# Autodesk Inventor assembly: Intake Full Assembly
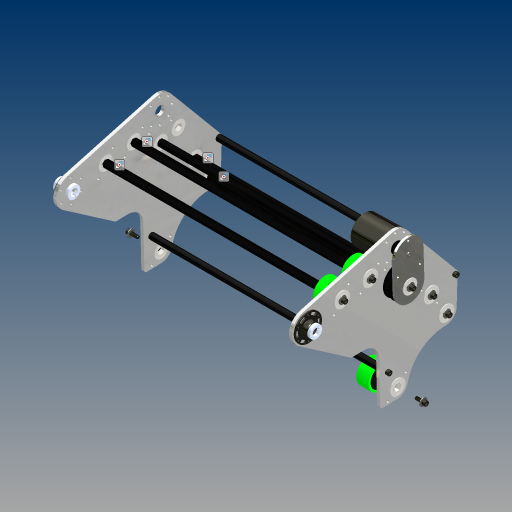
[picture p0: Inventor's stored thumbnail of the model, 512x512]
Saved by Autodesk Inventor 2024.3 (Build 283343000, 343)
## iProperties
Created: 2024-07-29
Part Number: Intake Full Assembly
Document SubType Name: Assembly
Designer: Kenji
Author: Kenji
## Documents named in this file (18)
- C:\Users\Kenji\Documents\GitHub\1622-2024-Summer-CAD-A-Thon\Intake\Intake Full Assembly.iam
- C:\Users\Kenji\Documents\GitHub\1622-2024-Summer-CAD-A-Thon\Intake\Intake Roller Plate.ipt
- C:\Users\Kenji\Documents\GitHub\1622-2024-Summer-CAD-A-Thon\COTS Library\Motion\Bearings\COTS_WCP-0783_1.125ODHexBearing.ipt
- C:\Users\Kenji\Documents\GitHub\1622-2024-Summer-CAD-A-Thon\Intake\Intake HexShaft 1.ipt
- C:\Users\Kenji\Documents\GitHub\1622-2024-Summer-CAD-A-Thon\COTS Library\Motion\Wheels\Compliant Wheels\2in compliant wheels\0.500in hex bore\COTS_am-3462_2indiameter_0.500inhexbore_durometer35A_CompliantWheel.ipt
- C:\Users\Kenji\Documents\GitHub\1622-2024-Summer-CAD-A-Thon\COTS Library\Motion\Wheels\Stealth Wheels\COTS_am-3155 2IN 500Hex Stealth Wheel.iam
- C:\Users\Kenji\Documents\GitHub\1622-2024-Summer-CAD-A-Thon\COTS Library\Structural Adapter\VersaHubs\COTS_217-2592_VersaHub.ipt
- C:\Users\Kenji\Documents\GitHub\1622-2024-Summer-CAD-A-Thon\Intake\Intake BeaterBar.ipt
- C:\Users\Kenji\Documents\GitHub\1622-2024-Summer-CAD-A-Thon\COTS Library\Fasteners\Bolts\Socket-Head\0.25-20\COTS_91251A539_Black-Oxide Alloy Steel Socket Head Screw (1).ipt
- C:\Users\Kenji\Documents\GitHub\1622-2024-Summer-CAD-A-Thon\COTS Library\Fasteners\Washers\COTS_90107A029_316 Stainless Steel Washer.ipt
- C:\Users\Kenji\Documents\GitHub\1622-2024-Summer-CAD-A-Thon\COTS Library\Fasteners\Shaft Collars\COTS_WCP-0799_0.5inchHexShaftCollar.ipt
- C:\Users\Kenji\Documents\GitHub\1622-2024-Summer-CAD-A-Thon\COTS Library\Motors\COTS_REV-21-1650-V1.1.ipt
- C:\Users\Kenji\Documents\GitHub\1622-2024-Summer-CAD-A-Thon\Intake\WCP-0076.ipt
- C:\Users\Kenji\Documents\GitHub\1622-2024-Summer-CAD-A-Thon\Intake\WCP-0990 (1).ipt
- C:\Users\Kenji\Documents\GitHub\1622-2024-Summer-CAD-A-Thon\Intake\WCP-0706.ipt
- C:\Users\Kenji\Documents\GitHub\1622-2024-Summer-CAD-A-Thon\Intake\WCP-0563.ipt
- C:\Users\Kenji\Documents\GitHub\1622-2024-Summer-CAD-A-Thon\Intake\Intake Hex Shaft 3.ipt
- C:\Users\Kenji\Documents\GitHub\1622-2024-Summer-CAD-A-Thon\Intake\Intake Pulley Cover 1.ipt
## Components (71 placed, 17 different names)
1. Intake Roller Plate:1 — Mate:293, Mate:294, Mate:295, Mate:296, Mate:297, Mate:298, Mate:299, Mate:302, Mate:303, Mate:304, Mate:306, Mate:307, Mate:308, Mate:310, Mate:311, Mate:312, Mate:313, Mate:314, Mate:315, Mate:316, Mate:317, Mate:318, Mate:319, Mate:320, Mate:321, Mate:364
2. Intake Roller Plate:2 — Mate:270, Mate:272, Mate:273, Mate:275, Mate:276, Mate:277, Mate:278, Mate:279, Mate:280, Mate:281, Mate:282, Mate:283, Mate:284, Mate:285, Mate:286, Mate:287, Mate:290, Mate:291, Mate:292, Mate:300, Mate:301, Mate:346, Mate:347, Mate:348
3. COTS_WCP-0783_1.125ODHexBearing:1 — Mate:25, Mate:276, Mate:283, Mate:329, Mate:340, Flush:10, Mate:355
4. COTS_WCP-0783_1.125ODHexBearing:2 — Mate:26, Mate:277, Mate:278, Mate:334, Mate:352, Mate:353
5. COTS_WCP-0783_1.125ODHexBearing:3 — Mate:272, Mate:280, Mate:332, Mate:337, Flush:11, Mate:358
6. COTS_WCP-0783_1.125ODHexBearing:4 — Mate:233, Mate:275, Mate:282, Mate:330, Mate:339, Flush:9, Mate:356
7. COTS_WCP-0783_1.125ODHexBearing:5 — Mate:270, Mate:271, Mate:279, Mate:333, Mate:336, Flush:12, Mate:357
8. COTS_WCP-0783_1.125ODHexBearing:6 — Mate:273, Mate:274, Mate:281, Mate:331, Mate:344, Mate:345
9. COTS_WCP-0783_1.125ODHexBearing:7 — Mate:135, Mate:319, Mate:320, Mate:326, Mate:360
10. COTS_WCP-0783_1.125ODHexBearing:8 — Mate:130, Mate:315, Mate:316, Mate:324, Mate:342, Mate:361
11. COTS_WCP-0783_1.125ODHexBearing:9 — Mate:134, Mate:317, Mate:318, Mate:325
12. COTS_WCP-0783_1.125ODHexBearing:10 — Mate:25, Mate:136, Mate:294, Mate:295, Mate:323, Mate:362
13. COTS_WCP-0783_1.125ODHexBearing:11 — Mate:26, Mate:132, Mate:144, Mate:293, Mate:321, Mate:328
14. COTS_WCP-0783_1.125ODHexBearing:12 — Mate:33, Mate:133, Mate:313, Mate:314, Mate:327, Mate:359
15. COTS_217-2592_VersaHub:2 — Mate:262, Mate:263, Mate:302, Mate:303, Mate:304, Mate:305
16. COTS_217-2592_VersaHub:3 — Mate:266, Mate:267, Mate:284, Mate:285, Mate:286
17. COTS_am-3462_2indiameter_0.500inhexbore_durometer35A_CompliantWheel:66 — Mate:136
18. COTS_am-3462_2indiameter_0.500inhexbore_durometer35A_CompliantWheel:24 — Mate:33, Mate:133
19. COTS_am-3462_2indiameter_0.500inhexbore_durometer35A_CompliantWheel:25 — Mate:134
20. COTS_am-3462_2indiameter_0.500inhexbore_durometer35A_CompliantWheel:53 — Mate:135
21. COTS_am-3462_2indiameter_0.500inhexbore_durometer35A_CompliantWheel:40 — Mate:130
22. COTS_am-3155 2IN 500Hex Stealth Wheel:7 [sub-assembly] — Mate:132, Mate:144
23. Intake BeaterBar:1 — Mate:251, Mate:297, Mate:298
24. Intake BeaterBar:2 — Mate:253, Mate:289, Mate:290, Mate:291, Mate:312
25. COTS_91251A539_Black-Oxide Alloy Steel Socket Head Screw (1):1 — Mate:212, Mate:213
26. COTS_91251A539_Black-Oxide Alloy Steel Socket Head Screw (1):2 — Mate:253, Mate:296
27. COTS_91251A539_Black-Oxide Alloy Steel Socket Head Screw (1):3 — Mate:214, Mate:215
28. COTS_91251A539_Black-Oxide Alloy Steel Socket Head Screw (1):4 — Mate:204, Mate:322
29. COTS_91251A539_Black-Oxide Alloy Steel Socket Head Screw (1):5 — Mate:195, Mate:196
30. COTS_91251A539_Black-Oxide Alloy Steel Socket Head Screw (1):6 — Mate:210, Mate:211
31. COTS_91251A539_Black-Oxide Alloy Steel Socket Head Screw (1):7 — Mate:189, Mate:190
32. COTS_91251A539_Black-Oxide Alloy Steel Socket Head Screw (1):8 — Mate:193, Mate:194
33. COTS_91251A539_Black-Oxide Alloy Steel Socket Head Screw (1):9 — Mate:251, Mate:300, Mate:301
34. COTS_91251A539_Black-Oxide Alloy Steel Socket Head Screw (1):10 — Mate:289, Mate:292
35. COTS_91251A539_Black-Oxide Alloy Steel Socket Head Screw (1):11 — Mate:216, Mate:217
36. COTS_91251A539_Black-Oxide Alloy Steel Socket Head Screw (1):12 — Mate:218, Mate:219
37. COTS_91251A539_Black-Oxide Alloy Steel Socket Head Screw (1):13 — Mate:299, Mate:307
38. COTS_91251A539_Black-Oxide Alloy Steel Socket Head Screw (1):14 — Mate:191, Mate:192
39. COTS_91251A539_Black-Oxide Alloy Steel Socket Head Screw (1):15 — Mate:187, Mate:188, Mate:233
40. COTS_91251A539_Black-Oxide Alloy Steel Socket Head Screw (1):16 — Mate:185, Mate:186
41. COTS_90107A029_316 Stainless Steel Washer:1 — Mate:212, Mate:213, Mate:326, Mate:360
42. COTS_90107A029_316 Stainless Steel Washer:2 — Mate:214, Mate:215, Mate:325, Mate:368
43. COTS_90107A029_316 Stainless Steel Washer:3 — Mate:193, Mate:194, Mate:271, Mate:333, Mate:357
44. COTS_90107A029_316 Stainless Steel Washer:4 — Mate:216, Mate:217, Mate:324, Mate:361
45. COTS_90107A029_316 Stainless Steel Washer:5 — Mate:187, Mate:188, Mate:330, Mate:356
46. COTS_90107A029_316 Stainless Steel Washer:6 — Mate:210, Mate:211, Mate:327, Mate:359
47. COTS_90107A029_316 Stainless Steel Washer:7 — Mate:204, Mate:322, Mate:328
48. COTS_90107A029_316 Stainless Steel Washer:8 — Mate:185, Mate:186, Mate:329, Mate:355
49. COTS_90107A029_316 Stainless Steel Washer:9 — Mate:218, Mate:219, Mate:323, Mate:362
50. COTS_90107A029_316 Stainless Steel Washer:10 — Mate:189, Mate:190, Mate:274, Mate:331
51. COTS_90107A029_316 Stainless Steel Washer:11 — Mate:195, Mate:196, Mate:334
52. COTS_90107A029_316 Stainless Steel Washer:12 — Mate:191, Mate:192, Mate:332, Mate:358
53. COTS_WCP-0799_0.5inchHexShaftCollar:1 — Mate:305, Mate:306
54. COTS_WCP-0799_0.5inchHexShaftCollar:2 — Mate:266, Mate:267, Mate:288
55. COTS_WCP-0799_0.5inchHexShaftCollar:3 — Mate:262, Mate:263
56. COTS_WCP-0799_0.5inchHexShaftCollar:4 — Mate:287, Mate:288
57. COTS_REV-21-1650-V1.1:2 — Mate:308, Mate:310, Mate:311, Mate:341, Angle:1, Flush:8
58. Intake HexShaft 1:2 — Mate:336, Flush:12
59. Intake HexShaft 1:3 — Mate:337, Flush:11
60. Intake HexShaft 1:4 — Mate:339, Flush:9
61. Intake HexShaft 1:6 — Mate:340, Flush:10
62. WCP-0076:1 — Mate:341, Angle:1, Mate:342, Flush:7
63. WCP-0990 (1):1 — Flush:7, Mate:367
64. WCP-0706:1 — Mate:344, Mate:345, Mate:354
65. WCP-0706:2 — Mate:346, Mate:349, Mate:350, Mate:351
66. COTS_WCP-0783_1.125ODHexBearing:13 — Mate:347, Mate:348, Mate:349
67. WCP-0563:1 — Mate:350, Mate:351
68. WCP-0563:2 — Mate:352, Mate:353
69. Intake Hex Shaft 3:1 — Mate:354, Flush:8, Mate:363, Flush:13
70. Intake Pulley Cover 1:1 — Mate:363, Mate:364, Mate:365, Mate:366
71. COTS_WCP-0783_1.125ODHexBearing:14 — Mate:365, Mate:366, Flush:13, Mate:367, Mate:368
## Relationships (143: Mate 135, Flush 7, Angle 1)
- Mate:25: COTS_WCP-0783_1.125ODHexBearing:1 ↔ COTS_WCP-0783_1.125ODHexBearing:10
- Mate:26: COTS_WCP-0783_1.125ODHexBearing:2 ↔ COTS_WCP-0783_1.125ODHexBearing:11
- Mate:33: COTS_WCP-0783_1.125ODHexBearing:12 ↔ COTS_am-3462_2indiameter_0.500inhexbore_durometer35A_CompliantWheel:24
- Mate:130 (15.24 mm): COTS_WCP-0783_1.125ODHexBearing:8 ↔ COTS_am-3462_2indiameter_0.500inhexbore_durometer35A_CompliantWheel:40
- Mate:132 (27.94 mm): COTS_WCP-0783_1.125ODHexBearing:11 ↔ COTS_am-3155 2IN 500Hex Stealth Wheel:7
- Mate:133 (15.24 mm): COTS_WCP-0783_1.125ODHexBearing:12 ↔ COTS_am-3462_2indiameter_0.500inhexbore_durometer35A_CompliantWheel:24
- Mate:134 (15.24 mm): COTS_WCP-0783_1.125ODHexBearing:9 ↔ COTS_am-3462_2indiameter_0.500inhexbore_durometer35A_CompliantWheel:25
- Mate:135 (15.24 mm): COTS_WCP-0783_1.125ODHexBearing:7 ↔ COTS_am-3462_2indiameter_0.500inhexbore_durometer35A_CompliantWheel:53
- Mate:136 (15.24 mm): COTS_WCP-0783_1.125ODHexBearing:10 ↔ COTS_am-3462_2indiameter_0.500inhexbore_durometer35A_CompliantWheel:66
- Mate:144: COTS_WCP-0783_1.125ODHexBearing:11 ↔ COTS_am-3155 2IN 500Hex Stealth Wheel:7
- Mate:185: COTS_91251A539_Black-Oxide Alloy Steel Socket Head Screw (1):16 ↔ COTS_90107A029_316 Stainless Steel Washer:8
- Mate:186: COTS_91251A539_Black-Oxide Alloy Steel Socket Head Screw (1):16 ↔ COTS_90107A029_316 Stainless Steel Washer:8
- Mate:187: COTS_91251A539_Black-Oxide Alloy Steel Socket Head Screw (1):15 ↔ COTS_90107A029_316 Stainless Steel Washer:5
- Mate:188: COTS_91251A539_Black-Oxide Alloy Steel Socket Head Screw (1):15 ↔ COTS_90107A029_316 Stainless Steel Washer:5
- Mate:189: COTS_91251A539_Black-Oxide Alloy Steel Socket Head Screw (1):7 ↔ COTS_90107A029_316 Stainless Steel Washer:10
- Mate:190: COTS_91251A539_Black-Oxide Alloy Steel Socket Head Screw (1):7 ↔ COTS_90107A029_316 Stainless Steel Washer:10
- Mate:191: COTS_91251A539_Black-Oxide Alloy Steel Socket Head Screw (1):14 ↔ COTS_90107A029_316 Stainless Steel Washer:12
- Mate:192: COTS_91251A539_Black-Oxide Alloy Steel Socket Head Screw (1):14 ↔ COTS_90107A029_316 Stainless Steel Washer:12
- Mate:193: COTS_91251A539_Black-Oxide Alloy Steel Socket Head Screw (1):8 ↔ COTS_90107A029_316 Stainless Steel Washer:3
- Mate:194: COTS_91251A539_Black-Oxide Alloy Steel Socket Head Screw (1):8 ↔ COTS_90107A029_316 Stainless Steel Washer:3
- Mate:195: COTS_91251A539_Black-Oxide Alloy Steel Socket Head Screw (1):5 ↔ COTS_90107A029_316 Stainless Steel Washer:11
- Mate:196: COTS_91251A539_Black-Oxide Alloy Steel Socket Head Screw (1):5 ↔ COTS_90107A029_316 Stainless Steel Washer:11
- Mate:204: COTS_91251A539_Black-Oxide Alloy Steel Socket Head Screw (1):4 ↔ COTS_90107A029_316 Stainless Steel Washer:7
- Mate:210: COTS_91251A539_Black-Oxide Alloy Steel Socket Head Screw (1):6 ↔ COTS_90107A029_316 Stainless Steel Washer:6
- Mate:211: COTS_91251A539_Black-Oxide Alloy Steel Socket Head Screw (1):6 ↔ COTS_90107A029_316 Stainless Steel Washer:6
- Mate:212: COTS_91251A539_Black-Oxide Alloy Steel Socket Head Screw (1):1 ↔ COTS_90107A029_316 Stainless Steel Washer:1
- Mate:213: COTS_91251A539_Black-Oxide Alloy Steel Socket Head Screw (1):1 ↔ COTS_90107A029_316 Stainless Steel Washer:1
- Mate:214: COTS_91251A539_Black-Oxide Alloy Steel Socket Head Screw (1):3 ↔ COTS_90107A029_316 Stainless Steel Washer:2
- Mate:215: COTS_91251A539_Black-Oxide Alloy Steel Socket Head Screw (1):3 ↔ COTS_90107A029_316 Stainless Steel Washer:2
- Mate:216: COTS_91251A539_Black-Oxide Alloy Steel Socket Head Screw (1):11 ↔ COTS_90107A029_316 Stainless Steel Washer:4
- Mate:217: COTS_91251A539_Black-Oxide Alloy Steel Socket Head Screw (1):11 ↔ COTS_90107A029_316 Stainless Steel Washer:4
- Mate:218: COTS_91251A539_Black-Oxide Alloy Steel Socket Head Screw (1):12 ↔ COTS_90107A029_316 Stainless Steel Washer:9
- Mate:219: COTS_91251A539_Black-Oxide Alloy Steel Socket Head Screw (1):12 ↔ COTS_90107A029_316 Stainless Steel Washer:9
- Mate:233: COTS_WCP-0783_1.125ODHexBearing:4 ↔ COTS_91251A539_Black-Oxide Alloy Steel Socket Head Screw (1):15
- Mate:251: Intake BeaterBar:1 ↔ COTS_91251A539_Black-Oxide Alloy Steel Socket Head Screw (1):9
- Mate:253: Intake BeaterBar:2 ↔ COTS_91251A539_Black-Oxide Alloy Steel Socket Head Screw (1):2
- Mate:262: COTS_217-2592_VersaHub:2 ↔ COTS_WCP-0799_0.5inchHexShaftCollar:3
- Mate:263: COTS_217-2592_VersaHub:2 ↔ COTS_WCP-0799_0.5inchHexShaftCollar:3
- Mate:266: COTS_217-2592_VersaHub:3 ↔ COTS_WCP-0799_0.5inchHexShaftCollar:2
- Mate:267: COTS_217-2592_VersaHub:3 ↔ COTS_WCP-0799_0.5inchHexShaftCollar:2
- Mate:270: Intake Roller Plate:2 ↔ COTS_WCP-0783_1.125ODHexBearing:5
- Mate:271: COTS_WCP-0783_1.125ODHexBearing:5 ↔ COTS_90107A029_316 Stainless Steel Washer:3
- Mate:272: Intake Roller Plate:2 ↔ COTS_WCP-0783_1.125ODHexBearing:3
- Mate:273: Intake Roller Plate:2 ↔ COTS_WCP-0783_1.125ODHexBearing:6
- Mate:274: COTS_WCP-0783_1.125ODHexBearing:6 ↔ COTS_90107A029_316 Stainless Steel Washer:10
- Mate:275: Intake Roller Plate:2 ↔ COTS_WCP-0783_1.125ODHexBearing:4
- Mate:276: Intake Roller Plate:2 ↔ COTS_WCP-0783_1.125ODHexBearing:1
- Mate:277: Intake Roller Plate:2 ↔ COTS_WCP-0783_1.125ODHexBearing:2
- Mate:278: Intake Roller Plate:2 ↔ COTS_WCP-0783_1.125ODHexBearing:2
- Mate:279: Intake Roller Plate:2 ↔ COTS_WCP-0783_1.125ODHexBearing:5
- Mate:280: Intake Roller Plate:2 ↔ COTS_WCP-0783_1.125ODHexBearing:3
- Mate:281: Intake Roller Plate:2 ↔ COTS_WCP-0783_1.125ODHexBearing:6
- Mate:282: Intake Roller Plate:2 ↔ COTS_WCP-0783_1.125ODHexBearing:4
- Mate:283: Intake Roller Plate:2 ↔ COTS_WCP-0783_1.125ODHexBearing:1
- Mate:284: Intake Roller Plate:2 ↔ COTS_217-2592_VersaHub:3
- Mate:285: Intake Roller Plate:2 ↔ COTS_217-2592_VersaHub:3
- Mate:286: Intake Roller Plate:2 ↔ COTS_217-2592_VersaHub:3
- Mate:287: Intake Roller Plate:2 ↔ COTS_WCP-0799_0.5inchHexShaftCollar:4
- Mate:288: COTS_WCP-0799_0.5inchHexShaftCollar:2 ↔ COTS_WCP-0799_0.5inchHexShaftCollar:4
- Mate:289: Intake BeaterBar:2 ↔ COTS_91251A539_Black-Oxide Alloy Steel Socket Head Screw (1):10
- Mate:290: Intake Roller Plate:2 ↔ Intake BeaterBar:2
- Mate:291: Intake Roller Plate:2 ↔ Intake BeaterBar:2
- Mate:292: Intake Roller Plate:2 ↔ COTS_91251A539_Black-Oxide Alloy Steel Socket Head Screw (1):10
- Mate:293: Intake Roller Plate:1 ↔ COTS_WCP-0783_1.125ODHexBearing:11
- Mate:294: Intake Roller Plate:1 ↔ COTS_WCP-0783_1.125ODHexBearing:10
- Mate:295: Intake Roller Plate:1 ↔ COTS_WCP-0783_1.125ODHexBearing:10
- Mate:296: Intake Roller Plate:1 ↔ COTS_91251A539_Black-Oxide Alloy Steel Socket Head Screw (1):2
- Mate:297: Intake Roller Plate:1 ↔ Intake BeaterBar:1
- Mate:298: Intake Roller Plate:1 ↔ Intake BeaterBar:1
- Mate:299: Intake Roller Plate:1 ↔ COTS_91251A539_Black-Oxide Alloy Steel Socket Head Screw (1):13
- Mate:300: Intake Roller Plate:2 ↔ COTS_91251A539_Black-Oxide Alloy Steel Socket Head Screw (1):9
- Mate:301: Intake Roller Plate:2 ↔ COTS_91251A539_Black-Oxide Alloy Steel Socket Head Screw (1):9
- Mate:302: Intake Roller Plate:1 ↔ COTS_217-2592_VersaHub:2
- Mate:303: Intake Roller Plate:1 ↔ COTS_217-2592_VersaHub:2
- Mate:304: Intake Roller Plate:1 ↔ COTS_217-2592_VersaHub:2
- Mate:305: COTS_217-2592_VersaHub:2 ↔ COTS_WCP-0799_0.5inchHexShaftCollar:1
- Mate:306: Intake Roller Plate:1 ↔ COTS_WCP-0799_0.5inchHexShaftCollar:1
- Mate:307: Intake Roller Plate:1 ↔ COTS_91251A539_Black-Oxide Alloy Steel Socket Head Screw (1):13
- Mate:308: Intake Roller Plate:1 ↔ COTS_REV-21-1650-V1.1:2
- Mate:310: Intake Roller Plate:1 ↔ COTS_REV-21-1650-V1.1:2
- Mate:311: Intake Roller Plate:1 ↔ COTS_REV-21-1650-V1.1:2
- Mate:312: Intake Roller Plate:1 ↔ Intake BeaterBar:2
- Mate:313: Intake Roller Plate:1 ↔ COTS_WCP-0783_1.125ODHexBearing:12
- Mate:314: Intake Roller Plate:1 ↔ COTS_WCP-0783_1.125ODHexBearing:12
- Mate:315: Intake Roller Plate:1 ↔ COTS_WCP-0783_1.125ODHexBearing:8
- Mate:316: Intake Roller Plate:1 ↔ COTS_WCP-0783_1.125ODHexBearing:8
- Mate:317: Intake Roller Plate:1 ↔ COTS_WCP-0783_1.125ODHexBearing:9
- Mate:318: Intake Roller Plate:1 ↔ COTS_WCP-0783_1.125ODHexBearing:9
- Mate:319: Intake Roller Plate:1 ↔ COTS_WCP-0783_1.125ODHexBearing:7
- Mate:320: Intake Roller Plate:1 ↔ COTS_WCP-0783_1.125ODHexBearing:7
- Mate:321: Intake Roller Plate:1 ↔ COTS_WCP-0783_1.125ODHexBearing:11
- Mate:322: COTS_91251A539_Black-Oxide Alloy Steel Socket Head Screw (1):4 ↔ COTS_90107A029_316 Stainless Steel Washer:7
- Mate:323: COTS_WCP-0783_1.125ODHexBearing:10 ↔ COTS_90107A029_316 Stainless Steel Washer:9
- Mate:324: COTS_WCP-0783_1.125ODHexBearing:8 ↔ COTS_90107A029_316 Stainless Steel Washer:4
- Mate:325: COTS_WCP-0783_1.125ODHexBearing:9 ↔ COTS_90107A029_316 Stainless Steel Washer:2
- Mate:326: COTS_WCP-0783_1.125ODHexBearing:7 ↔ COTS_90107A029_316 Stainless Steel Washer:1
- Mate:327: COTS_WCP-0783_1.125ODHexBearing:12 ↔ COTS_90107A029_316 Stainless Steel Washer:6
- Mate:328: COTS_WCP-0783_1.125ODHexBearing:11 ↔ COTS_90107A029_316 Stainless Steel Washer:7
- Mate:329: COTS_WCP-0783_1.125ODHexBearing:1 ↔ COTS_90107A029_316 Stainless Steel Washer:8
- Mate:330: COTS_WCP-0783_1.125ODHexBearing:4 ↔ COTS_90107A029_316 Stainless Steel Washer:5
- Mate:331: COTS_WCP-0783_1.125ODHexBearing:6 ↔ COTS_90107A029_316 Stainless Steel Washer:10
- Mate:332: COTS_WCP-0783_1.125ODHexBearing:3 ↔ COTS_90107A029_316 Stainless Steel Washer:12
- Mate:333: COTS_WCP-0783_1.125ODHexBearing:5 ↔ COTS_90107A029_316 Stainless Steel Washer:3
- Mate:334: COTS_WCP-0783_1.125ODHexBearing:2 ↔ COTS_90107A029_316 Stainless Steel Washer:11
- Mate:336: COTS_WCP-0783_1.125ODHexBearing:5 ↔ Intake HexShaft 1:2
- Mate:337: COTS_WCP-0783_1.125ODHexBearing:3 ↔ Intake HexShaft 1:3
- Mate:339: COTS_WCP-0783_1.125ODHexBearing:4 ↔ Intake HexShaft 1:4
- Mate:340: COTS_WCP-0783_1.125ODHexBearing:1 ↔ Intake HexShaft 1:6
- Mate:341: COTS_REV-21-1650-V1.1:2 ↔ WCP-0076:1
- Angle:1 (0 deg): COTS_REV-21-1650-V1.1:2 ↔ WCP-0076:1
- Mate:342: COTS_WCP-0783_1.125ODHexBearing:8 ↔ WCP-0076:1
- Flush:7: WCP-0076:1 ↔ WCP-0990 (1):1
- Mate:344: COTS_WCP-0783_1.125ODHexBearing:6 ↔ WCP-0706:1
- Mate:345: COTS_WCP-0783_1.125ODHexBearing:6 ↔ WCP-0706:1
- Mate:346: Intake Roller Plate:2 ↔ WCP-0706:2
- Mate:347: Intake Roller Plate:2 ↔ COTS_WCP-0783_1.125ODHexBearing:13
- Mate:348: Intake Roller Plate:2 ↔ COTS_WCP-0783_1.125ODHexBearing:13
- Mate:349: WCP-0706:2 ↔ COTS_WCP-0783_1.125ODHexBearing:13
- Mate:350: WCP-0706:2 ↔ WCP-0563:1
- Mate:351: WCP-0706:2 ↔ WCP-0563:1
- Mate:352: COTS_WCP-0783_1.125ODHexBearing:2 ↔ WCP-0563:2
- Mate:353: COTS_WCP-0783_1.125ODHexBearing:2 ↔ WCP-0563:2
- Mate:354: WCP-0706:1 ↔ Intake Hex Shaft 3:1
- Flush:8: COTS_REV-21-1650-V1.1:2 ↔ Intake Hex Shaft 3:1
- Flush:9: COTS_WCP-0783_1.125ODHexBearing:4 ↔ Intake HexShaft 1:4
- Flush:10: COTS_WCP-0783_1.125ODHexBearing:1 ↔ Intake HexShaft 1:6
- Flush:11: COTS_WCP-0783_1.125ODHexBearing:3 ↔ Intake HexShaft 1:3
- Flush:12: COTS_WCP-0783_1.125ODHexBearing:5 ↔ Intake HexShaft 1:2
- Mate:355: COTS_WCP-0783_1.125ODHexBearing:1 ↔ COTS_90107A029_316 Stainless Steel Washer:8
- Mate:356: COTS_WCP-0783_1.125ODHexBearing:4 ↔ COTS_90107A029_316 Stainless Steel Washer:5
- Mate:357: COTS_WCP-0783_1.125ODHexBearing:5 ↔ COTS_90107A029_316 Stainless Steel Washer:3
- Mate:358: COTS_WCP-0783_1.125ODHexBearing:3 ↔ COTS_90107A029_316 Stainless Steel Washer:12
- Mate:359: COTS_WCP-0783_1.125ODHexBearing:12 ↔ COTS_90107A029_316 Stainless Steel Washer:6
- Mate:360: COTS_WCP-0783_1.125ODHexBearing:7 ↔ COTS_90107A029_316 Stainless Steel Washer:1
- Mate:361: COTS_WCP-0783_1.125ODHexBearing:8 ↔ COTS_90107A029_316 Stainless Steel Washer:4
- Mate:362: COTS_WCP-0783_1.125ODHexBearing:10 ↔ COTS_90107A029_316 Stainless Steel Washer:9
- Mate:363: Intake Hex Shaft 3:1 ↔ Intake Pulley Cover 1:1
- Mate:364: Intake Roller Plate:1 ↔ Intake Pulley Cover 1:1
- Mate:365: Intake Pulley Cover 1:1 ↔ COTS_WCP-0783_1.125ODHexBearing:14
- Mate:366: Intake Pulley Cover 1:1 ↔ COTS_WCP-0783_1.125ODHexBearing:14
- Flush:13: Intake Hex Shaft 3:1 ↔ COTS_WCP-0783_1.125ODHexBearing:14
- Mate:367: WCP-0990 (1):1 ↔ COTS_WCP-0783_1.125ODHexBearing:14
- Mate:368: COTS_90107A029_316 Stainless Steel Washer:2 ↔ COTS_WCP-0783_1.125ODHexBearing:14
